# Autodesk Inventor assembly: EL2-.300
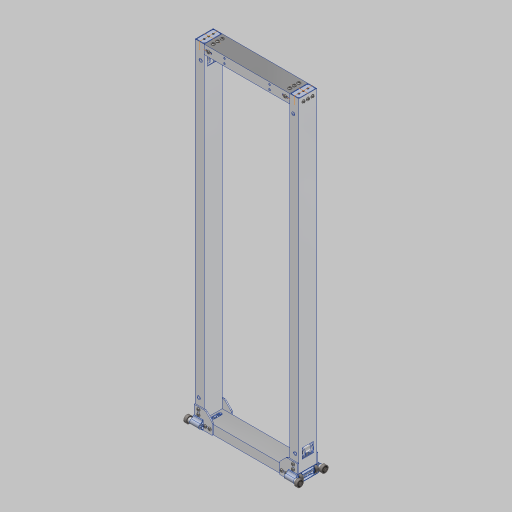
[picture p0: Inventor's stored thumbnail of the model, 512x512]
Saved by Autodesk Inventor 2023.5 (Build 275446000, 446)
## iProperties
Created: 2025-01-11
Part Number: EL2-.300
Document SubType Name: Assembly
Designer: mavericks
Mass: 1994.64 g
Surface Area: 8276.32 cm^2
Volume: 714.95 cm^3
Density: 2.7899 g/cm^3
Author: mavericks
## Documents named in this file (11)
- C:\Users\slick\OneDrive\Desktop\2025-ReefScape---CAD\Elevator\EL2\EL2-.300.iam
- C:\Users\slick\OneDrive\Desktop\2025-ReefScape---CAD\Elevator\EL2\EL2-004.ipt
- C:\Users\slick\OneDrive\Desktop\2025-ReefScape---CAD\COMMON PARTS\WCP Elevator parts\WCP-0199\WCP-0199.iam
- C:\Users\slick\OneDrive\Desktop\2025-ReefScape---CAD\Elevator\EL2\EL2-006.ipt
- C:\Users\slick\OneDrive\Desktop\2025-ReefScape---CAD\Elevator\EL2\EL2-005.ipt
- C:\Users\slick\OneDrive\Desktop\2025-ReefScape---CAD\Elevator\EL2\EL2-400.iam
- C:\Users\slick\OneDrive\Desktop\2025-ReefScape---CAD\Elevator\EL2\EL2-010.ipt
- C:\Users\slick\OneDrive\Desktop\2025-ReefScape---CAD\Elevator\EL2\EL2-011.ipt
- C:\Users\slick\OneDrive\Desktop\2025-ReefScape---CAD\Content Center\en-US\U UNC 2605\Unbrako - 10 x 5_16 - 24(10).ipt
- C:\Users\slick\OneDrive\Desktop\2025-ReefScape---CAD\Content Center\en-US\U UNC 2605\Unbrako - 10 x 1 - 24(10).ipt
- C:\Users\slick\OneDrive\Desktop\2025-ReefScape---CAD\Content Center\en-US\U UNC 2605\Unbrako - 10 x 3_8 - 32(10).ipt
## Components (54 placed, 10 different names)
1. EL2-004:1 — Flush:1, Flush:2, Mate:1, Insert:3, Flush:12, Symmetry:1, Insert:4, Insert:6, Insert:8, Insert:13, Insert:14, Insert:25, Insert:29, Insert:30, Insert:32, Flush:14, Insert:52, Insert:53, Insert:54
2. WCP-0199:1 [sub-assembly] — Flush:1, Flush:2, Mate:1
3. EL2-011:1 — Flush:8, Insert:9, Insert:10, Insert:11, Insert:12, Insert:15, Insert:16, Insert:22, Insert:23, Insert:24, Insert:26, Insert:27, Insert:28
4. EL2-004:2 — Symmetry:1, Insert:5, Insert:7, Insert:17, Insert:18, Insert:19, Insert:20, Insert:21, Insert:31, Insert:49, Insert:50, Insert:51
5. WCP-0199:2 [sub-assembly] — Flush:8
6. EL2-006:3 — Flush:12, Flush:13, Insert:65, Insert:72, Insert:73, Insert:80, Insert:81, Insert:82, Insert:83, Insert:84, Insert:85, Insert:86, Insert:87, Insert:88, Insert:89, Insert:90, Insert:91, Insert:92
7. EL2-005:3
8. EL2-005:4 — Insert:3
9. EL2-400:1 [sub-assembly] — Insert:5
10. EL2-400:2 [sub-assembly] — Insert:4
11. EL2-400:3 [sub-assembly] — Insert:6
12. EL2-400:4 [sub-assembly] — Insert:7
13. EL2-010:1 — Insert:8, Insert:9, Insert:11, Insert:12, Insert:13, Insert:14, Mate:10, Mate:11, Mate:16, Mate:17, Mate:18, Mate:19, Mate:20, Mate:21
14. EL2-010:2 — Insert:10, Insert:15, Insert:16, Insert:17, Insert:18, Insert:33, Insert:36, Insert:37, Insert:38
15. EL2-010:3 — Insert:25, Insert:26, Insert:27, Insert:28, Insert:29, Insert:30, Insert:46, Insert:47, Insert:48
16. EL2-010:4 — Insert:19, Insert:20, Insert:21, Insert:22, Insert:23, Insert:24, Insert:40, Insert:41, Insert:42
17. EL2-005:5 — Flush:13, Insert:31
18. EL2-005:6 — Insert:32, Flush:14
19. Unbrako UNC Hex Socket Button Cap - Inch 10 x 5/16:1 — Insert:33
20. Unbrako UNC Hex Socket Button Cap - Inch 10 x 5/16:4 — Insert:36
21. Unbrako UNC Hex Socket Button Cap - Inch 10 x 5/16:5 — Insert:37
22. Unbrako UNC Hex Socket Button Cap - Inch 10 x 5/16:6 — Insert:38
23. Unbrako UNC Hex Socket Button Cap - Inch 10 x 5/16:8 — Insert:40
24. Unbrako UNC Hex Socket Button Cap - Inch 10 x 5/16:9 — Insert:41
25. Unbrako UNC Hex Socket Button Cap - Inch 10 x 5/16:10 — Insert:42
26. Unbrako UNC Hex Socket Button Cap - Inch 10 x 5/16:14 — Insert:46
27. Unbrako UNC Hex Socket Button Cap - Inch 10 x 5/16:15 — Insert:47
28. Unbrako UNC Hex Socket Button Cap - Inch 10 x 5/16:16 — Insert:48
29. Unbrako UNC Hex Socket Button Cap - Inch 10 x 5/16:19 — Mate:10, Mate:11
30. Unbrako UNC Hex Socket Button Cap - Inch 10 x 5/16:22 — Mate:16, Mate:17
31. Unbrako UNC Hex Socket Button Cap - Inch 10 x 5/16:23 — Mate:18, Mate:19
32. Unbrako UNC Hex Socket Button Cap - Inch 10 x 5/16:24 — Mate:20, Mate:21
33. Unbrako UNC Hex Socket Button Cap - Inch 10 x 1:1 — Insert:49
34. Unbrako UNC Hex Socket Button Cap - Inch 10 x 1:2 — Insert:50
35. Unbrako UNC Hex Socket Button Cap - Inch 10 x 1:3 — Insert:51
36. Unbrako UNC Hex Socket Button Cap - Inch 10 x 1:4 — Insert:52
37. Unbrako UNC Hex Socket Button Cap - Inch 10 x 1:5 — Insert:53
38. Unbrako UNC Hex Socket Button Cap - Inch 10 x 1:6 — Insert:54
39. Unbrako UNC Hex Socket Button Cap - Inch 10 x 3/8:1 — Insert:65
40. Unbrako UNC Hex Socket Button Cap - Inch 10 x 3/8:8 — Insert:72
41. Unbrako UNC Hex Socket Button Cap - Inch 10 x 3/8:9 — Insert:73
42. Unbrako UNC Hex Socket Button Cap - Inch 10 x 3/8:16 — Insert:80
43. Unbrako UNC Hex Socket Button Cap - Inch 10 x 3/8:17 — Insert:81
44. Unbrako UNC Hex Socket Button Cap - Inch 10 x 3/8:18 — Insert:82
45. Unbrako UNC Hex Socket Button Cap - Inch 10 x 3/8:19 — Insert:83
46. Unbrako UNC Hex Socket Button Cap - Inch 10 x 3/8:20 — Insert:84
47. Unbrako UNC Hex Socket Button Cap - Inch 10 x 3/8:21 — Insert:85
48. Unbrako UNC Hex Socket Button Cap - Inch 10 x 3/8:22 — Insert:86
49. Unbrako UNC Hex Socket Button Cap - Inch 10 x 3/8:23 — Insert:87
50. Unbrako UNC Hex Socket Button Cap - Inch 10 x 3/8:24 — Insert:88
51. Unbrako UNC Hex Socket Button Cap - Inch 10 x 3/8:25 — Insert:89
52. Unbrako UNC Hex Socket Button Cap - Inch 10 x 3/8:26 — Insert:90
53. Unbrako UNC Hex Socket Button Cap - Inch 10 x 3/8:27 — Insert:91
54. Unbrako UNC Hex Socket Button Cap - Inch 10 x 3/8:28 — Insert:92
## Relationships (87: Insert 62, Mate 13, Flush 11, Symmetry 1)
- Flush:1: EL2-004:1 ↔ WCP-0199:1
- Flush:2: EL2-004:1 ↔ WCP-0199:1
- Mate:1: EL2-004:1 ↔ WCP-0199:1
- [Flush]: EL2-004:2 ↔ WCP-0199:2
- [Flush]: EL2-004:2 ↔ WCP-0199:2
- [Mate]: EL2-004:2 ↔ WCP-0199:2
- Flush:8: EL2-011:1 ↔ WCP-0199:2
- [Flush]: EL2-006:3 ↔ EL2-005:3
- [Flush]: EL2-006:3 ↔ EL2-005:3
- [Mate]: EL2-006:3 ↔ EL2-005:3
- [Mate]: EL2-006:3 ↔ EL2-005:4
- [Mate]: EL2-006:3 ↔ EL2-005:4
- [Flush]: EL2-006:3 ↔ EL2-005:4
- Insert:3: EL2-004:1 ↔ EL2-005:4
- Flush:12: EL2-004:1 ↔ EL2-006:3
- Symmetry:1: EL2-004:1 ↔ EL2-004:2
- Insert:4: EL2-004:1 ↔ EL2-400:2
- Insert:5: EL2-004:2 ↔ EL2-400:1
- Insert:6: EL2-004:1 ↔ EL2-400:3
- Insert:7: EL2-004:2 ↔ EL2-400:4
- Insert:8: EL2-004:1 ↔ EL2-010:1
- Insert:9: EL2-011:1 ↔ EL2-010:1
- Insert:10: EL2-011:1 ↔ EL2-010:2
- Insert:11: EL2-011:1 ↔ EL2-010:1
- Insert:12: EL2-011:1 ↔ EL2-010:1
- Insert:13: EL2-004:1 ↔ EL2-010:1
- Insert:14: EL2-004:1 ↔ EL2-010:1
- Insert:15: EL2-011:1 ↔ EL2-010:2
- Insert:16: EL2-011:1 ↔ EL2-010:2
- Insert:17: EL2-004:2 ↔ EL2-010:2
- Insert:18: EL2-004:2 ↔ EL2-010:2
- Insert:19: EL2-004:2 ↔ EL2-010:4
- Insert:20: EL2-004:2 ↔ EL2-010:4
- Insert:21: EL2-004:2 ↔ EL2-010:4
- Insert:22: EL2-011:1 ↔ EL2-010:4
- Insert:23: EL2-011:1 ↔ EL2-010:4
- Insert:24: EL2-011:1 ↔ EL2-010:4
- Insert:25: EL2-004:1 ↔ EL2-010:3
- Insert:26: EL2-011:1 ↔ EL2-010:3
- Insert:27: EL2-011:1 ↔ EL2-010:3
- Insert:28: EL2-011:1 ↔ EL2-010:3
- Insert:29: EL2-004:1 ↔ EL2-010:3
- Insert:30: EL2-004:1 ↔ EL2-010:3
- Flush:13: EL2-006:3 ↔ EL2-005:5
- Insert:31: EL2-004:2 ↔ EL2-005:5
- Insert:32: EL2-004:1 ↔ EL2-005:6
- Flush:14: EL2-004:1 ↔ EL2-005:6
- Insert:33: EL2-010:2 ↔ Unbrako UNC Hex Socket Button Cap - Inch 10 x 5/16:1
- Insert:36: EL2-010:2 ↔ Unbrako UNC Hex Socket Button Cap - Inch 10 x 5/16:4
- Insert:37: EL2-010:2 ↔ Unbrako UNC Hex Socket Button Cap - Inch 10 x 5/16:5
- Insert:38: EL2-010:2 ↔ Unbrako UNC Hex Socket Button Cap - Inch 10 x 5/16:6
- Insert:40: EL2-010:4 ↔ Unbrako UNC Hex Socket Button Cap - Inch 10 x 5/16:8
- Insert:41: EL2-010:4 ↔ Unbrako UNC Hex Socket Button Cap - Inch 10 x 5/16:9
- Insert:42: EL2-010:4 ↔ Unbrako UNC Hex Socket Button Cap - Inch 10 x 5/16:10
- Insert:46: EL2-010:3 ↔ Unbrako UNC Hex Socket Button Cap - Inch 10 x 5/16:14
- Insert:47: EL2-010:3 ↔ Unbrako UNC Hex Socket Button Cap - Inch 10 x 5/16:15
- Insert:48: EL2-010:3 ↔ Unbrako UNC Hex Socket Button Cap - Inch 10 x 5/16:16
- Mate:10: EL2-010:1 ↔ Unbrako UNC Hex Socket Button Cap - Inch 10 x 5/16:19
- Mate:11: EL2-010:1 ↔ Unbrako UNC Hex Socket Button Cap - Inch 10 x 5/16:19
- Mate:16: EL2-010:1 ↔ Unbrako UNC Hex Socket Button Cap - Inch 10 x 5/16:22
- Mate:17: EL2-010:1 ↔ Unbrako UNC Hex Socket Button Cap - Inch 10 x 5/16:22
- Mate:18: EL2-010:1 ↔ Unbrako UNC Hex Socket Button Cap - Inch 10 x 5/16:23
- Mate:19: EL2-010:1 ↔ Unbrako UNC Hex Socket Button Cap - Inch 10 x 5/16:23
- Mate:20: EL2-010:1 ↔ Unbrako UNC Hex Socket Button Cap - Inch 10 x 5/16:24
- Mate:21: EL2-010:1 ↔ Unbrako UNC Hex Socket Button Cap - Inch 10 x 5/16:24
- Insert:49: EL2-004:2 ↔ Unbrako UNC Hex Socket Button Cap - Inch 10 x 1:1
- Insert:50: EL2-004:2 ↔ Unbrako UNC Hex Socket Button Cap - Inch 10 x 1:2
- Insert:51: EL2-004:2 ↔ Unbrako UNC Hex Socket Button Cap - Inch 10 x 1:3
- Insert:52: EL2-004:1 ↔ Unbrako UNC Hex Socket Button Cap - Inch 10 x 1:4
- Insert:53: EL2-004:1 ↔ Unbrako UNC Hex Socket Button Cap - Inch 10 x 1:5
- Insert:54: EL2-004:1 ↔ Unbrako UNC Hex Socket Button Cap - Inch 10 x 1:6
- Insert:65: EL2-006:3 ↔ Unbrako UNC Hex Socket Button Cap - Inch 10 x 3/8:1
- Insert:72: EL2-006:3 ↔ Unbrako UNC Hex Socket Button Cap - Inch 10 x 3/8:8
- Insert:73: EL2-006:3 ↔ Unbrako UNC Hex Socket Button Cap - Inch 10 x 3/8:9
- Insert:80: EL2-006:3 ↔ Unbrako UNC Hex Socket Button Cap - Inch 10 x 3/8:16
- Insert:81: EL2-006:3 ↔ Unbrako UNC Hex Socket Button Cap - Inch 10 x 3/8:17
- Insert:82: EL2-006:3 ↔ Unbrako UNC Hex Socket Button Cap - Inch 10 x 3/8:18
- Insert:83: EL2-006:3 ↔ Unbrako UNC Hex Socket Button Cap - Inch 10 x 3/8:19
- Insert:84: EL2-006:3 ↔ Unbrako UNC Hex Socket Button Cap - Inch 10 x 3/8:20
- Insert:85: EL2-006:3 ↔ Unbrako UNC Hex Socket Button Cap - Inch 10 x 3/8:21
- Insert:86: EL2-006:3 ↔ Unbrako UNC Hex Socket Button Cap - Inch 10 x 3/8:22
- Insert:87: EL2-006:3 ↔ Unbrako UNC Hex Socket Button Cap - Inch 10 x 3/8:23
- Insert:88: EL2-006:3 ↔ Unbrako UNC Hex Socket Button Cap - Inch 10 x 3/8:24
- Insert:89: EL2-006:3 ↔ Unbrako UNC Hex Socket Button Cap - Inch 10 x 3/8:25
- Insert:90: EL2-006:3 ↔ Unbrako UNC Hex Socket Button Cap - Inch 10 x 3/8:26
- Insert:91: EL2-006:3 ↔ Unbrako UNC Hex Socket Button Cap - Inch 10 x 3/8:27
- Insert:92: EL2-006:3 ↔ Unbrako UNC Hex Socket Button Cap - Inch 10 x 3/8:28
## Named parameters: d11_d0 = 0 mm, d12_d1 = 0 mm, d13_d2 = 0 mm, d16_d3 = 0 mm, d17_d4 = 0 mm, d18_d5 = 0 mm, d19_d6 = 0 mm, d20_d7 = 0 mm, d21_d8 = 0 mm
